# Autodesk Inventor assembly: SCARA
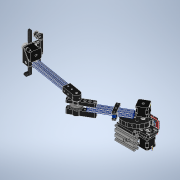
[picture p0: Inventor's stored thumbnail of the model, 180x180]
Saved by Autodesk Inventor 2022 (Build 260153000, 153)
## iProperties
Created: 2022-03-02
Part Number: SCARA
Document SubType Name: Assembly
Designer: JK
Author: JK
## Documents named in this file (6)
- C:\Users\FabLab\Desktop\JK\SCARA-3DP\Parts\SCARA.iam
- C:\Users\FabLab\Desktop\JK\SCARA-3DP\Parts\Shoulder\Shoulder base.iam
- C:\Users\FabLab\Desktop\JK\SCARA-3DP\Parts\Elbow\Elbow assembly.iam
- C:\Users\FabLab\Desktop\JK\SCARA-3DP\Parts\Z axis\Z assembly.iam
- C:\Users\FabLab\Desktop\JK\SCARA-3DP\Parts\Electronics\Electronics.iam
- C:\Users\FabLab\Desktop\JK\SCARA-3DP\Parts\25T0397-001.ipt
## Components (5 placed, 5 different names)
1. Shoulder base:1 [sub-assembly] — Coincidencia:5, Coincidencia:6, Nivelación:4, Coincidencia:17, Nivelación:5, Nivelación:6
2. Elbow assembly:1 [sub-assembly] — Coincidencia:5, Coincidencia:6, Coincidencia:14, Nivelación:4, Coincidencia:16, Coincidencia:18
3. Z assembly:1 [sub-assembly] — Nivelación:3, Coincidencia:14, Coincidencia:16, Coincidencia:18
4. Electronics:1 [sub-assembly] — Coincidencia:17, Nivelación:5, Nivelación:6
5. 25T0397-001:1 — Nivelación:3
## Relationships (10: Mate 6, Flush 4)
- Coincidencia:5 [Mate]: Shoulder base:1 ↔ Elbow assembly:1
- Coincidencia:6 [Mate] (-30 mm): Shoulder base:1 ↔ Elbow assembly:1
- Nivelación:3 [Flush] (5 mm): Z assembly:1 ↔ 25T0397-001:1
- Coincidencia:14 [Mate] (0.15 mm): Elbow assembly:1 ↔ Z assembly:1
- Nivelación:4 [Flush]: Shoulder base:1 ↔ Elbow assembly:1
- Coincidencia:16 [Mate]: Elbow assembly:1 ↔ Z assembly:1
- Coincidencia:17 [Mate]: Shoulder base:1 ↔ Electronics:1
- Nivelación:5 [Flush] (1 mm): Shoulder base:1 ↔ Electronics:1
- Nivelación:6 [Flush]: Shoulder base:1 ↔ Electronics:1
- Coincidencia:18 [Mate]: Elbow assembly:1 ↔ Z assembly:1
